# Autodesk Inventor assembly: Assembly1.Tube and Pipe Runs
(part 2 of 2)
Elbow45Key: v3#2769403e-a4fd-4a4c-8e4c-659ea845bd78#2
_ComponentInfo: <CS><C N="Pipe" R="2.400000" IR="2.040000" PL="PL" PN="JIS K 6741 Pipe VP 40"><CO N="1"><FE V="0"/><FD V="1"/><ET V="Jointed"/><NS V="M40"/><MA  V="4.000000"/><MI V="0.800000"/><WP X="0.000000" Y="0.000000" Z="0.000000"/><WA X="-1.000000" Y="0.000000" Z="0.000000"/></CO><CO N="2"><FE  V="0"/><FD V="0"/><ET V="Jointed"/><NS V="M40"/><MA V="4.000000"/><MI V="0.800000"/><WP X="-25.000000" Y="0.000000" Z="0.000000"/><WA X="-1.000000"  Y="0.000000" Z="0.000000"/></CO></C><C N="Coupling" CW="4.700000"><CO N="1"><FE V="1"/><FD V="1"/><ET V="Jointed"/><NS V="M40"/><MA V="2.200000"/><MI  V="0.440000"/><WP X="0.000000" Y="0.000000" Z="0.000000"/><WA X="1.000000" Y="0.000000" Z="0.000000"/></CO><CO N="2"><FE V="1"/><FD V="0"/><ET  V="Jointed"/><NS V="M40"/><MA V="2.200000"/><MI V="0.440000"/><WP X="4.700000" Y="0.000000" Z="0.000000"/><WA X="1.000000" Y="0.000000"  Z="0.000000"/></CO></C><C N="Elbow90" ER="2.700000" S1="4.900000" S2="4.900000" D1="2.200000" D2="2.200000"><CO N="1"><FE V="1"/><FD V="1"/><ET  V="Jointed"/><NS V="M40"/><MA V="2.200000"/><MI V="0.440000"/><WP X="4.900000" Y="0.000000" Z="4.900000"/><WA X="-1.000000" Y="0.000000"  Z="0.000000"/></CO><CO N="2"><FE V="1"/><FD V="0"/><ET V="Jointed"/><NS V="M40"/><MA V="2.200000"/><MI V="0.440000"/><WP X="0.000000" Y="0.000000"  Z="0.000000"/><WA X="0.000000" Y="0.000000" Z="-1.000000"/></CO></C><C N="Elbow45" ER="3.379899" S1="3.600000" S2="3.600000" D1="2.200000"  D2="2.200000"><CO N="1"><FE V="1"/><FD V="1"/><ET V="Jointed"/><NS V="M40"/><MA V="2.200000"/><MI V="0.440000"/><WP X="2.545584" Y="0.000000"  Z="6.145584"/><WA X="-0.707107" Y="0.000000" Z="-0.707107"/></CO><CO N="2"><FE V="1"/><FD V="0"/><ET V="Jointed"/><NS V="M40"/><MA V="2.200000"/><MI  V="0.440000"/><WP X="0.000000" Y="0.000000" Z="0.000000"/><WA X="0.000000" Y="0.000000" Z="-1.000000"/></CO></C></CS>
Name: DIN 8062/DIN 8063 - Jointed PVC-U Pipe and Fittings
Schedule: 6.3
PipeKey: v3#3d294dc7-89c3-4c37-a0ae-28c15a73bfd0#13
CouplingKey: v3#3edf83e2-464b-4b31-84c5-c329ffbf2a4f#5
Elbow90Key: v3#fbd68fd5-590c-4cb5-8c20-9e9bdd396a04#5
Elbow45Key: v3#2f597a97-b15b-49d4-87cb-7bfe69eb62ee#5
_ComponentInfo: <CS><C N="Pipe" R="2.000000" IR="1.700000" PL="PL" PN="DIN 8062 Pipe 40 x 3"><CO N="1"><FE V="0"/><FD V="0"/><ET V="Jointed"/><NS V="M40"/><MA  V="8.000000"/><MI V="1.600000"/><WP X="25.000000" Y="0.000000" Z="0.000000"/><WA X="1.000000" Y="0.000000" Z="0.000000"/></CO><CO N="2"><FE  V="0"/><FD V="1"/><ET V="Jointed"/><NS V="M40"/><MA V="8.000000"/><MI V="1.600000"/><WP X="0.000000" Y="0.000000" Z="0.000000"/><WA X="1.000000"  Y="0.000000" Z="0.000000"/></CO></C><C N="Coupling" CW="5.500000"><CO N="1"><FE V="1"/><FD V="1"/><ET V="Jointed"/><NS V="M40"/><MA V="2.600000"/><MI  V="0.520000"/><WP X="0.000000" Y="0.000000" Z="0.000000"/><WA X="1.000000" Y="0.000000" Z="0.000000"/></CO><CO N="2"><FE V="1"/><FD V="0"/><ET  V="Jointed"/><NS V="M40"/><MA V="2.600000"/><MI V="0.520000"/><WP X="5.500000" Y="0.000000" Z="0.000000"/><WA X="1.000000" Y="0.000000"  Z="0.000000"/></CO></C><C N="Elbow90" ER="8.000000" S1="10.600000" S2="10.600000" D1="2.600000" D2="2.600000"><CO N="1"><FE V="1"/><FD V="0"/><ET  V="Jointed"/><NS V="M40"/><MA V="2.600000"/><MI V="0.520000"/><WP X="10.600000" Y="0.000000" Z="10.600000"/><WA X="1.000000" Y="0.000000"  Z="-0.000000"/></CO><CO N="2"><FE V="1"/><FD V="0"/><ET V="Jointed"/><NS V="M40"/><MA V="2.600000"/><MI V="0.520000"/><WP X="0.000000" Y="0.000000"  Z="-0.000000"/><WA X="-0.000000" Y="0.000000" Z="-1.000000"/></CO></C><C N="Elbow45" ER="2.293503" S1="3.550000" S2="3.550000" D1="2.600000"  D2="2.600000"><CO N="1"><FE V="1"/><FD V="0"/><ET V="Jointed"/><NS V="M40"/><MA V="2.600000"/><MI V="0.520000"/><WP X="2.510229" Y="0.000000"  Z="6.060229"/><WA X="0.707107" Y="0.000000" Z="0.707107"/></CO><CO N="2"><FE V="1"/><FD V="0"/><ET V="Jointed"/><NS V="M40"/><MA V="2.600000"/><MI  V="0.520000"/><WP X="0.000000" Y="0.000000" Z="0.000000"/><WA X="-0.000000" Y="0.000000" Z="-1.000000"/></CO></C></CS>
Name: ISO 4065-ISO 3633 - PVC Pipe and Fittings
Schedule: S40
IntermediateSegmentsMax: 2540 mm
TerminationSegmentsMax: 2540 mm
PipeKey: v3#4f84f716-5ba0-45ef-967a-c32c3d7345ce#70
CouplingKey: v3#b06656e5-2b55-488c-bcf0-6a90c79c4683#2
Elbow90Key: v3#17490b17-1dd8-40fc-8de7-1a70c3bab2d7#1
Elbow45Key: v3#421a8b99-1721-409a-bc3b-c00889561754#1
_ComponentInfo: <CS><C N="Pipe" R="2.000000" IR="1.950000" PL="PL" PN="ISO 4065 Pipe 40 x 0.5 S40"><CO N="1"><FE V="0"/><FD V="0"/><ET V="Jointed"/><NS V="M40"/><MA  V="6.000000"/><MI V="1.200000"/><WP X="25.000000" Y="0.000000" Z="0.000000"/><WA X="1.000000" Y="0.000000" Z="0.000000"/></CO><CO N="2"><FE  V="0"/><FD V="1"/><ET V="Jointed"/><NS V="M40"/><MA V="6.000000"/><MI V="1.200000"/><WP X="0.000000" Y="0.000000" Z="0.000000"/><WA X="1.000000"  Y="0.000000" Z="0.000000"/></CO></C><C N="Coupling" CW="7.660000"><CO N="1"><FE V="1"/><FD V="1"/><ET V="Jointed"/><NS V="M40"/><MA V="3.830000"/><MI  V="0.766000"/><WP X="-0.000000" Y="0.000000" Z="0.000000"/><WA X="-1.000000" Y="0.000000" Z="0.000000"/></CO><CO N="2"><FE V="1"/><FD V="0"/><ET  V="Jointed"/><NS V="M40"/><MA V="3.830000"/><MI V="0.766000"/><WP X="-7.660000" Y="0.000000" Z="0.000000"/><WA X="-1.000000" Y="0.000000"  Z="0.000000"/></CO></C><C N="Elbow90" ER="3.850394" S1="7.450394" S2="7.450394" D1="3.600000" D2="3.600000"><CO N="1"><FE V="1"/><FD V="1"/><ET  V="Jointed"/><NS V="M40"/><MA V="3.600000"/><MI V="0.720000"/><WP X="7.450394" Y="0.000000" Z="7.450394"/><WA X="-1.000000" Y="0.000000"  Z="0.000000"/></CO><CO N="2"><FE V="1"/><FD V="0"/><ET V="Jointed"/><NS V="M40"/><MA V="3.600000"/><MI V="0.720000"/><WP X="-0.000000" Y="0.000000"  Z="0.000000"/><WA X="0.000000" Y="0.000000" Z="-1.000000"/></CO></C><C N="Elbow45" ER="5.674352" S1="5.950394" S2="5.950394" D1="3.600000"  D2="3.600000"><CO N="1"><FE V="1"/><FD V="1"/><ET V="Jointed"/><NS V="M40"/><MA V="3.600000"/><MI V="0.720000"/><WP X="4.207564" Y="0.000000"  Z="10.157957"/><WA X="-0.707107" Y="0.000000" Z="-0.707107"/></CO><CO N="2"><FE V="1"/><FD V="0"/><ET V="Jointed"/><NS V="M40"/><MA V="3.600000"/><MI  V="0.720000"/><WP X="-0.000000" Y="0.000000" Z="0.000000"/><WA X="0.000000" Y="0.000000" Z="-1.000000"/></CO></C></CS>
count: 33
Refkey_Axis1_Context: 2|0|0|0|1|0|0|0|
Refkey_Axis1: 6|0|0|0|44|0|0|0|78|0|65|0|77|0|69|0|83|0|10|0|67|0|111|0|108|0|111|0|114|0|115|0|10|0|49|0|58|0|10|0|10|0|69|0|78|0|68|0|10|0|0|0|
Refkey_Axis2_Context: 2|0|0|0|1|0|0|0|
Refkey_Axis2: 6|0|0|0|88|0|0|0|78|0|65|0|77|0|69|0|83|0|10|0|67|0|111|0|108|0|111|0|114|0|115|0|10|0|49|0|58|0|82|0|111|0|117|0|116|0|101|0|32|0|85|0|73|0|32|0|84|0|111|0|111|0|108|0|32|0|40|0|65|0|120|0|105|0|115|0|32|0|50|0|41|0|10|0|10|0|69|0|78|0|68|0|10|0|0|0|
Refkey_Axis3_Context: 2|0|0|0|1|0|0|0|
Refkey_Axis3: 6|0|0|0|88|0|0|0|78|0|65|0|77|0|69|0|83|0|10|0|67|0|111|0|108|0|111|0|114|0|115|0|10|0|49|0|58|0|82|0|111|0|117|0|116|0|101|0|32|0|85|0|73|0|32|0|84|0|111|0|111|0|108|0|32|0|40|0|65|0|120|0|105|0|115|0|32|0|51|0|41|0|10|0|10|0|69|0|78|0|68|0|10|0|0|0|
Refkey_Ext_Context: 2|0|0|0|1|0|0|0|
Refkey_Ext: 6|0|0|0|92|0|0|0|78|0|65|0|77|0|69|0|83|0|10|0|67|0|111|0|108|0|111|0|114|0|115|0|10|0|49|0|58|0|82|0|111|0|117|0|116|0|101|0|32|0|85|0|73|0|32|0|84|0|111|0|111|0|108|0|32|0|40|0|69|0|120|0|116|0|101|0|110|0|100|0|101|0|114|0|41|0|10|0|10|0|69|0|78|0|68|0|10|0|0|0|
Refkey_Snap_Context: 2|0|0|0|1|0|0|0|
Refkey_Snap: 6|0|0|0|84|0|0|0|78|0|65|0|77|0|69|0|83|0|10|0|67|0|111|0|108|0|111|0|114|0|115|0|10|0|49|0|58|0|82|0|111|0|117|0|116|0|101|0|32|0|85|0|73|0|32|0|84|0|111|0|111|0|108|0|32|0|40|0|83|0|110|0|97|0|112|0|41|0|10|0|10|0|69|0|78|0|68|0|10|0|0|0|
Name: Hydraulic Hose - No Fittings
_ComponentInfo: <CS><C N="Pipe" R="1.117600" OR="1.117600" IR="0.635000" PL="PL" PartType="" SymKey="" PN="Parker Hydraulic Hose - No Skive 1/2"><CO N="1"><FE V="0"/><FD V="0"/><ET V="Hose - Permanent"/><NS V="1/2"/><MA V="2.540000"/><MI V="0.508000"/><WP X="12.700000" Y="0.000000" Z="0.000000"/><WA X="1.000000" Y="0.000000" Z="0.000000"/></CO><CO N="2"><FE V="0"/><FD V="1"/><ET V="Hose - Permanent"/><NS V="1/2"/><MA V="2.540000"/><MI V="0.508000"/><WP X="0.000000" Y="0.000000" Z="0.000000"/><WA X="1.000000" Y="0.000000" Z="0.000000"/></CO></C></CS>
SuppressStartFitting: True
SuppressEndFitting: True
Author: halli
## Documents named in this file (2)
- D:\14gabillah\12gabillah\Rangkuman Engineering\Mechanical Engineering\practice-engineering-drawing (main branch)\Piping\Pakai Inventor\Assembly1.Tube and Pipe Runs.iam
- D:\14gabillah\12gabillah\Rangkuman Engineering\Mechanical Engineering\practice-engineering-drawing (main branch)\Piping\Piping Project 1\Route 2\Assembly1.Run01.iam
## Components (1 placed, 1 different names)
1. Run 01 [sub-assembly]
